# Autodesk Inventor assembly: Assembly
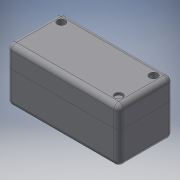
[picture p0: Inventor's stored thumbnail of the model, 180x180]
Saved by Autodesk Inventor 2019 (Build 230136000, 136)
## iProperties
Created: 2019-04-30
Part Number: Assembly
Document SubType Name: Assembly
Designer: Henry
Author: Henry
## Documents named in this file (4)
- D:\Projects\DogWifi\Inventor\Assembly.iam
- D:\Projects\DogWifi\Inventor\PCB.ipt
- D:\Projects\DogWifi\Inventor\BottomcaseV2.ipt
- D:\Projects\DogWifi\Inventor\Topcase.ipt
## Components (3 placed, 3 different names)
1. BottomcaseV2:1 — Mate:1, Mate:2, Mate:3, Mate:4, Mate:5, Mate:6
2. PCB:1 — Mate:1, Mate:2, Mate:3
3. Topcase:1 — Mate:4, Mate:5, Mate:6
## Relationships (6: Mate 6)
- Mate:1 (1 mm): BottomcaseV2:1 ↔ PCB:1
- Mate:2 (1 mm): BottomcaseV2:1 ↔ PCB:1
- Mate:3: BottomcaseV2:1 ↔ PCB:1
- Mate:4: BottomcaseV2:1 ↔ Topcase:1
- Mate:5 (-2 mm): BottomcaseV2:1 ↔ Topcase:1
- Mate:6 (-2 mm): BottomcaseV2:1 ↔ Topcase:1
